# Autodesk Inventor assembly: 付け根ロール_1
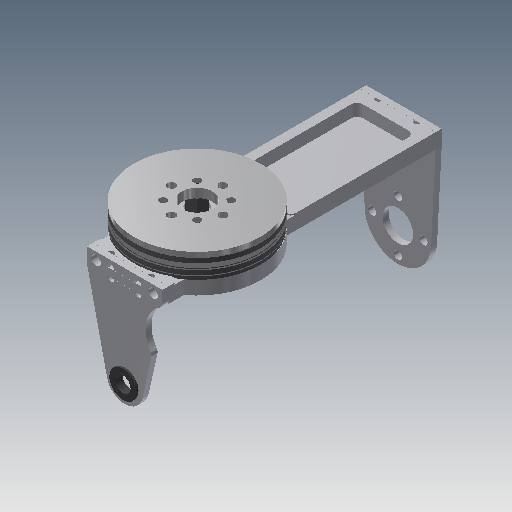
[picture p0: Inventor's stored thumbnail of the model, 512x512]
Saved by Autodesk Inventor 2017.3 (Build 213256000, 256)
## iProperties
Created: 2016-05-01
Part Number: 付け根ロール_1
Document SubType Name: Assembly
Designer: hiroaki
Mass: 38.2338 g
Surface Area: 222.3 cm^2
Volume: 16.8041 cm^3
Density: 2.27527 g/cm^3
Author: hiroaki
## Documents named in this file (9)
- C:\Users\haya\Desktop\GankenKun0_5\下半身\付け根ロール\付け根ロール_1.iam
- C:\Users\haya\Desktop\GankenKun0_5\下半身\付け根ロール\付け根ロール_メインフレーム_1_1.ipt
- C:\Users\haya\Desktop\GankenKun0_5\下半身\付け根ロール\付け根ロール_サブフレーム_1_1.ipt
- C:\Users\haya\Desktop\GankenKun0_5\下半身\付け根ロール\付け根ロール_サブフレーム_1_2.ipt
- C:\Users\haya\Desktop\GankenKun0_5\既製品\NSK_RB_MF85ZZ\MF85ZZ.iam
- C:\Users\haya\Desktop\GankenKun0_5\既製品\BA2542\core_BA2542.ipt
- C:\Users\haya\Desktop\GankenKun0_5\下半身\付け根ロール\付け根ロール_サブフレーム_1_4.ipt
- C:\Users\haya\Desktop\GankenKun0_5\既製品\BA2542\washer_BA2542.ipt
- C:\Users\haya\Desktop\GankenKun0_5\既製品\SLCG5_5-6.ipt
## Components (12 placed, 8 different names)
1. 付け根ロール_メインフレーム_1_1:1 — 挿入:2, 挿入:5, 挿入:13, 挿入:14, 挿入:29, 挿入:31, 挿入:32, 挿入:33, 挿入:34
2. 付け根ロール_サブフレーム_1_1:1 — 挿入:5, 挿入:14
3. 付け根ロール_サブフレーム_1_2:1 — 挿入:1, 挿入:2, 挿入:13
4. MF85ZZ:1 [sub-assembly] — 挿入:1
5. core_BA2542:1 — 挿入:30
6. core_BA2542:2 — 挿入:24
7. 付け根ロール_サブフレーム_1_4:1 — 挿入:24, 挿入:35, 挿入:36, 挿入:37
8. washer_BA2542:1 — 挿入:29, 挿入:30
9. SLCG5_5-6:1 — 挿入:31, 挿入:35
10. SLCG5_5-6:2 — 挿入:32, 挿入:36
11. SLCG5_5-6:3 — 挿入:33
12. SLCG5_5-6:4 — 挿入:34, 挿入:37
## Relationships (15: Insert 15)
- 挿入:1 [Insert]: 付け根ロール_サブフレーム_1_2:1 ↔ MF85ZZ:1
- 挿入:2 [Insert]: 付け根ロール_メインフレーム_1_1:1 ↔ 付け根ロール_サブフレーム_1_2:1
- 挿入:5 [Insert]: 付け根ロール_メインフレーム_1_1:1 ↔ 付け根ロール_サブフレーム_1_1:1
- 挿入:13 [Insert]: 付け根ロール_メインフレーム_1_1:1 ↔ 付け根ロール_サブフレーム_1_2:1
- 挿入:14 [Insert]: 付け根ロール_メインフレーム_1_1:1 ↔ 付け根ロール_サブフレーム_1_1:1
- 挿入:24 [Insert]: core_BA2542:2 ↔ 付け根ロール_サブフレーム_1_4:1
- 挿入:29 [Insert]: 付け根ロール_メインフレーム_1_1:1 ↔ washer_BA2542:1
- 挿入:30 [Insert]: core_BA2542:1 ↔ washer_BA2542:1
- 挿入:31 [Insert]: 付け根ロール_メインフレーム_1_1:1 ↔ SLCG5_5-6:1
- 挿入:32 [Insert]: 付け根ロール_メインフレーム_1_1:1 ↔ SLCG5_5-6:2
- 挿入:33 [Insert]: 付け根ロール_メインフレーム_1_1:1 ↔ SLCG5_5-6:3
- 挿入:34 [Insert]: 付け根ロール_メインフレーム_1_1:1 ↔ SLCG5_5-6:4
- 挿入:35 [Insert]: 付け根ロール_サブフレーム_1_4:1 ↔ SLCG5_5-6:1
- 挿入:36 [Insert]: 付け根ロール_サブフレーム_1_4:1 ↔ SLCG5_5-6:2
- 挿入:37 [Insert]: 付け根ロール_サブフレーム_1_4:1 ↔ SLCG5_5-6:4
